# Autodesk Inventor assembly: 1 Pound Flamethrower Assembly
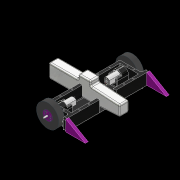
[picture p0: Inventor's stored thumbnail of the model, 180x180]
Saved by Autodesk Inventor 2022 (Build 260153000, 153)
## iProperties
Created: 2022-05-16
Part Number: 1 Pound Flamethrower Assembly
Document SubType Name: Assembly
Designer: tandu
Author: tandu
## Documents named in this file (7)
- C:\Users\tandu\Documents\GrabCAD\1 Pound Flamethrower\1 Pound Flamethrower Assembly.iam
- C:\Users\tandu\Documents\GrabCAD\1 Pound Flamethrower\90417A126_Phillips Rounded Head Thread-Forming Screws.ipt
- C:\Users\tandu\Documents\GrabCAD\1 Pound Flamethrower\CorrectSizeWheelsIThink.ipt
- C:\Users\tandu\Documents\GrabCAD\1 Pound Flamethrower\FingerTech_Silver_Spark_223350.ipt
- C:\Users\tandu\Documents\GrabCAD\1 Pound Flamethrower\Flamethrower TPU 22 Chassis.ipt
- C:\Users\tandu\Documents\GrabCAD\1 Pound Flamethrower\WedgeUHMWPiece.ipt
- C:\Users\tandu\Documents\GrabCAD\1 Pound Flamethrower\FlamethrowerModule.ipt
## Components (12 placed, 6 different names)
1. 90417A126_Phillips Rounded Head Thread-Forming Screws:1 — Insert:12
2. CorrectSizeWheelsIThink:1 — Insert:8
3. FingerTech_Silver_Spark_223350:1 — Insert:5, Mate:1
4. Flamethrower TPU 22 Chassis:1 — Flush:1, Flush:2, Flush:3, Insert:1, Insert:2, Insert:5, Insert:6, Mate:1, Mate:2, Insert:7, Insert:8, Insert:9, Insert:10, Insert:11, Insert:12, Insert:13, Insert:14, Mate:3
5. WedgeUHMWPiece:1 — Insert:1, Insert:2
6. WedgeUHMWPiece:2 — Insert:13, Insert:14
7. CorrectSizeWheelsIThink:2 — Insert:7
8. FingerTech_Silver_Spark_223350:2 — Insert:6, Mate:2
9. 90417A126_Phillips Rounded Head Thread-Forming Screws:2 — Insert:11
10. 90417A126_Phillips Rounded Head Thread-Forming Screws:3 — Insert:10
11. 90417A126_Phillips Rounded Head Thread-Forming Screws:4 — Insert:9
12. FlamethrowerModule:1 — Mate:3
## Relationships (18: Insert 12, Flush 3, Mate 3)
- Flush:1: Flamethrower TPU 22 Chassis:1
- Flush:2: Flamethrower TPU 22 Chassis:1
- Flush:3: Flamethrower TPU 22 Chassis:1
- Insert:1: Flamethrower TPU 22 Chassis:1 ↔ WedgeUHMWPiece:1
- Insert:2: Flamethrower TPU 22 Chassis:1 ↔ WedgeUHMWPiece:1
- Insert:5: FingerTech_Silver_Spark_223350:1 ↔ Flamethrower TPU 22 Chassis:1
- Insert:6: Flamethrower TPU 22 Chassis:1 ↔ FingerTech_Silver_Spark_223350:2
- Mate:1: FingerTech_Silver_Spark_223350:1 ↔ Flamethrower TPU 22 Chassis:1
- Mate:2: Flamethrower TPU 22 Chassis:1 ↔ FingerTech_Silver_Spark_223350:2
- Insert:7: Flamethrower TPU 22 Chassis:1 ↔ CorrectSizeWheelsIThink:2
- Insert:8: CorrectSizeWheelsIThink:1 ↔ Flamethrower TPU 22 Chassis:1
- Insert:9: Flamethrower TPU 22 Chassis:1 ↔ 90417A126_Phillips Rounded Head Thread-Forming Screws:4
- Insert:10: Flamethrower TPU 22 Chassis:1 ↔ 90417A126_Phillips Rounded Head Thread-Forming Screws:3
- Insert:11: Flamethrower TPU 22 Chassis:1 ↔ 90417A126_Phillips Rounded Head Thread-Forming Screws:2
- Insert:12: 90417A126_Phillips Rounded Head Thread-Forming Screws:1 ↔ Flamethrower TPU 22 Chassis:1
- Insert:13: Flamethrower TPU 22 Chassis:1 ↔ WedgeUHMWPiece:2
- Insert:14: Flamethrower TPU 22 Chassis:1 ↔ WedgeUHMWPiece:2
- Mate:3: Flamethrower TPU 22 Chassis:1 ↔ FlamethrowerModule:1
